# Autodesk Inventor assembly: Wheel Insert Inner Context
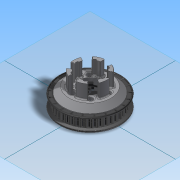
[picture p0: Inventor's stored thumbnail of the model, 180x180]
Saved by Autodesk Inventor 2014 SP2 (Build 180246200, 246)
## iProperties
Created: 2014-05-22
Part Number: Wheel Insert Inner Context
Document SubType Name: Assembly
Designer: dliu
Author: dliu
## Documents named in this file (4)
- C:\Users\dliu\Dropbox\dbhome\electric-longboard\dliu\Wheel Insert\Wheel Insert InnerAdapter Context.iam
- C:\Users\dliu\Dropbox\dbhome\electric-longboard\dliu\Wheel Insert\Wheel Insert Sketch.ipt
- C:\Users\dliu\Dropbox\dbhome\electric-longboard\dliu\Wheel Insert\Wheel Insert InnerAdapter.ipt
- C:\Users\dliu\Dropbox\dbhome\electric-longboard\dliu\Pulleys\ThinVersaPulley.iam
## Components (3 placed, 3 different names)
1. Wheel Insert Sketch:1 — Mate:2, Mate:4, Mate:5
2. Wheel Insert InnerAdapter:1 — Flush:3, Mate:5, Mate:6, Mate:7
3. ThinVersaPulley:1 [sub-assembly] — Mate:6, Mate:7
## Relationships (6: Mate 5, Flush 1)
- Mate:2: Wheel Insert Sketch:1
- Mate:4: Wheel Insert Sketch:1
- Flush:3: Wheel Insert InnerAdapter:1
- Mate:5: Wheel Insert Sketch:1 ↔ Wheel Insert InnerAdapter:1
- Mate:6: Wheel Insert InnerAdapter:1 ↔ ThinVersaPulley:1
- Mate:7: Wheel Insert InnerAdapter:1 ↔ ThinVersaPulley:1
